# Autodesk Inventor assembly: JewlArm
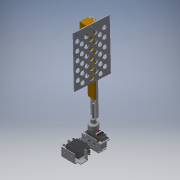
[picture p0: Inventor's stored thumbnail of the model, 180x180]
Saved by Autodesk Inventor 2017 (Build 210142000, 142)
## iProperties
Created: 2017-10-12
Part Number: JewlArm
Document SubType Name: Assembly
Designer: User
Author: User
## Documents named in this file (7)
- C:\Robotics\CAD\2017-18_CAD\Miscellaneous\JewlArm.iam
- C:\Robotics\CAD\COTSParts\Tetrix\Tetrix servo 180.ipt
- C:\Robotics\CAD\COTSParts\Tetrix\Tetrix bracket - single servo.ipt
- C:\Robotics\CAD\2017-18_CAD\FlapperSlapperPlate.ipt
- C:\Robotics\CAD\2017-18_CAD\FlapperSlapper.ipt
- C:\Robotics\CAD\COTSParts\Bosch Extrusion\Bosch 20x20 10in half.ipt
- C:\Robotics\CAD\2017-18_CAD\20X20Connector.ipt
## Components (8 placed, 6 different names)
1. Tetrix servo 180:1 — Mate:11, Mate:12, Mate:13, Mate:21, Mate:22
2. Tetrix servo 180:2 — Mate:10, Mate:18, Mate:19, Mate:20
3. Tetrix bracket - single servo:1 — Mate:18, Mate:19, Mate:20, Flush:1, Flush:2
4. Tetrix bracket - single servo:2 — Mate:10, Mate:11, Mate:12, Mate:13, Flush:1, Flush:2
5. FlapperSlapperPlate:1 — Mate:27, Flush:4, Flush:5
6. FlapperSlapper:1 — Mate:21, Mate:22, Mate:24, Tangent:1, Tangent:2
7. Bosch 20x20 10in half:1 — Mate:24, Tangent:1, Tangent:2, Flush:3, Mate:25, Mate:26
8. 20X20Connector:1 — Flush:3, Mate:25, Mate:26, Mate:27, Flush:4, Flush:5
## Relationships (20: Mate 13, Flush 5, Tangent 2)
- Mate:10 (10.668 mm): Tetrix servo 180:2 ↔ Tetrix bracket - single servo:2
- Mate:11: Tetrix servo 180:1 ↔ Tetrix bracket - single servo:2
- Mate:12: Tetrix servo 180:1 ↔ Tetrix bracket - single servo:2
- Mate:13: Tetrix servo 180:1 ↔ Tetrix bracket - single servo:2
- Mate:18 (10.16 mm): Tetrix servo 180:2 ↔ Tetrix bracket - single servo:1
- Mate:19: Tetrix servo 180:2 ↔ Tetrix bracket - single servo:1
- Mate:20: Tetrix servo 180:2 ↔ Tetrix bracket - single servo:1
- Flush:1 (6.35 mm): Tetrix bracket - single servo:1 ↔ Tetrix bracket - single servo:2
- Flush:2: Tetrix bracket - single servo:1 ↔ Tetrix bracket - single servo:2
- Mate:21: Tetrix servo 180:1 ↔ FlapperSlapper:1
- Mate:22: Tetrix servo 180:1 ↔ FlapperSlapper:1
- Mate:24 (-31.75 mm): FlapperSlapper:1 ↔ Bosch 20x20 10in half:1
- Tangent:1: FlapperSlapper:1 ↔ Bosch 20x20 10in half:1
- Tangent:2: FlapperSlapper:1 ↔ Bosch 20x20 10in half:1
- Flush:3: Bosch 20x20 10in half:1 ↔ 20X20Connector:1
- Mate:25: Bosch 20x20 10in half:1 ↔ 20X20Connector:1
- Mate:26: Bosch 20x20 10in half:1 ↔ 20X20Connector:1
- Mate:27: FlapperSlapperPlate:1 ↔ 20X20Connector:1
- Flush:4: FlapperSlapperPlate:1 ↔ 20X20Connector:1
- Flush:5 (38.1 mm): FlapperSlapperPlate:1 ↔ 20X20Connector:1
